# Autodesk Inventor assembly: Motorhalterung_Foerderband.ipt
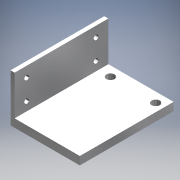
[picture p0: Inventor's stored thumbnail of the model, 180x180]
Saved by Autodesk Inventor 2018 (Build 220112000, 112)
## iProperties
Created: 2018-03-26
Part Number: Motorhalterung_Foerderband.ipt
Material: Generisch
Document SubType Name: Assembly
Designer: Julian
Author: Julian
## Documents named in this file (4)
- C:\Users\Julian\Desktop\Schule\5AHME\Diplomarbeit\Git\fuettr_prototype\Mechanical\Inventorskizzen\Motorhalterung_Foerderband.ipt.iam
- C:\Users\Julian\Desktop\Schule\5AHME\Diplomarbeit\Git\fuettr_prototype\Mechanical\Inventorskizzen\Motorhalterung_Grundplatte.ipt
- C:\Users\Julian\Desktop\Schule\5AHME\Diplomarbeit\Git\fuettr_prototype\Mechanical\Inventorskizzen\Motorhalterung_Stützleiste.ipt
- C:\Users\Julian\Documents\Inventor\Content Center Files\R2018\de-DE\ISO 4762(1)\DIN EN ISO 4762 - M5 x 12.ipt
## Components (5 placed, 3 different names)
1. Motorhalterung_Grundplatte:1 — Starr:2
2. Motorhalterung_Stützleiste:1 — Starr:2, Starr:3, Starr:4, Starr:5
3. DIN EN ISO 4762 M5 x 12:1 — Starr:3
4. DIN EN ISO 4762 M5 x 12:2 — Starr:4
5. DIN EN ISO 4762 M5 x 12:3 — Starr:5
## Relationships (4: WeldJoint 4)
- Starr:2 [WeldJoint]: Motorhalterung_Grundplatte:1 ↔ Motorhalterung_Stützleiste:1
- Starr:3 [WeldJoint]: Motorhalterung_Stützleiste:1 ↔ DIN EN ISO 4762 M5 x 12:1
- Starr:4 [WeldJoint]: Motorhalterung_Stützleiste:1 ↔ DIN EN ISO 4762 M5 x 12:2
- Starr:5 [WeldJoint]: Motorhalterung_Stützleiste:1 ↔ DIN EN ISO 4762 M5 x 12:3
